# Autodesk Inventor assembly: BaseAssemblyMk1
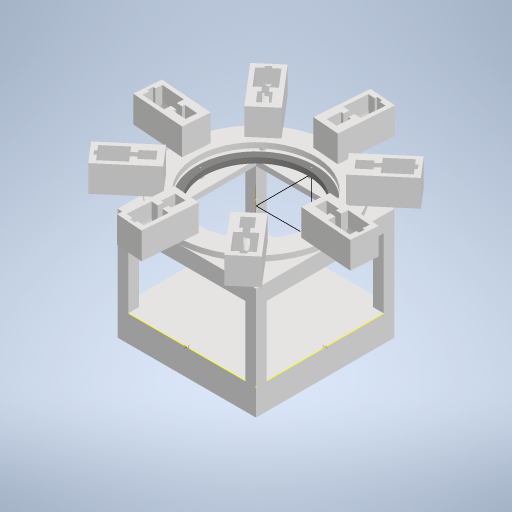
[picture p0: Inventor's stored thumbnail of the model, 512x512]
Saved by Autodesk Inventor 2023 (Build 270158000, 158)
## iProperties
Created: 2023-03-23
Part Number: BaseAssemblyMk1
Document SubType Name: Assembly
Designer: czapa
Author: czapa
## Documents named in this file (6)
- C:\Users\czapa\OneDrive\Documents\GitHub\S.P.I.C.E\3D Models\Version1\BaseAssemblyMk1.iam
- C:\Users\czapa\OneDrive\Documents\GitHub\S.P.I.C.E\3D Models\Version1\BaseMk1.ipt
- C:\Users\czapa\OneDrive\Documents\GitHub\S.P.I.C.E\3D Models\Version1\InnerBearingTable.ipt
- C:\Users\czapa\OneDrive\Documents\GitHub\S.P.I.C.E\3D Models\Version1\OuterBearingTable.ipt
- C:\Users\czapa\OneDrive\Documents\GitHub\S.P.I.C.E\3D Models\Version1\TableCover.ipt
- C:\Users\czapa\OneDrive\Documents\GitHub\S.P.I.C.E\3D Models\dcmotor_housing.ipt
## Components (12 placed, 5 different names)
1. BaseMk1:1 — Mate:1, Mate:2, Mate:3
2. InnerBearingTable:1 — Mate:1, Mate:2, Mate:3, Mate:4, Flush:1
3. OuterBearingTable:1 — Mate:4, Flush:1, Mate:5, Mate:6, Mate:7
4. TableCover:1 — Mate:5, Mate:6, Mate:7, Mate:8, Mate:9, Mate:10, Flush:2, Flush:3, Flush:4, Flush:5, Flush:6, Flush:7, Flush:8, Mate:11, Mate:12, Mate:13, Mate:14, Mate:15, Mate:16, Mate:17, Mate:18, Mate:19, Mate:20, Mate:21, Mate:22, Mate:23, Mate:24
5. dcmotor_housing:1 — Mate:8, Mate:9, Mate:10
6. dcmotor_housing:2 — Flush:2, Mate:11, Mate:18
7. dcmotor_housing:3 — Flush:5, Mate:12, Mate:21
8. dcmotor_housing:4 — Flush:8, Mate:14, Mate:19
9. dcmotor_housing:5 — Flush:6, Mate:16, Mate:22
10. dcmotor_housing:6 — Flush:3, Mate:13, Mate:23
11. dcmotor_housing:7 — Flush:4, Mate:17, Mate:20
12. dcmotor_housing:8 — Flush:7, Mate:15, Mate:24
## Relationships (32: Mate 24, Flush 8)
- Mate:1: BaseMk1:1 ↔ InnerBearingTable:1
- Mate:2: BaseMk1:1 ↔ InnerBearingTable:1
- Mate:3: BaseMk1:1 ↔ InnerBearingTable:1
- Mate:4: InnerBearingTable:1 ↔ OuterBearingTable:1
- Flush:1: InnerBearingTable:1 ↔ OuterBearingTable:1
- Mate:5: OuterBearingTable:1 ↔ TableCover:1
- Mate:6: OuterBearingTable:1 ↔ TableCover:1
- Mate:7: OuterBearingTable:1 ↔ TableCover:1
- Mate:8: TableCover:1 ↔ dcmotor_housing:1
- Mate:9: TableCover:1 ↔ dcmotor_housing:1
- Mate:10: TableCover:1 ↔ dcmotor_housing:1
- Flush:2: TableCover:1 ↔ dcmotor_housing:2
- Flush:3: TableCover:1 ↔ dcmotor_housing:6
- Flush:4: TableCover:1 ↔ dcmotor_housing:7
- Flush:5: TableCover:1 ↔ dcmotor_housing:3
- Flush:6: TableCover:1 ↔ dcmotor_housing:5
- Flush:7: TableCover:1 ↔ dcmotor_housing:8
- Flush:8: TableCover:1 ↔ dcmotor_housing:4
- Mate:11: TableCover:1 ↔ dcmotor_housing:2
- Mate:12: TableCover:1 ↔ dcmotor_housing:3
- Mate:13: TableCover:1 ↔ dcmotor_housing:6
- Mate:14: TableCover:1 ↔ dcmotor_housing:4
- Mate:15: TableCover:1 ↔ dcmotor_housing:8
- Mate:16: TableCover:1 ↔ dcmotor_housing:5
- Mate:17: TableCover:1 ↔ dcmotor_housing:7
- Mate:18: TableCover:1 ↔ dcmotor_housing:2
- Mate:19: TableCover:1 ↔ dcmotor_housing:4
- Mate:20: TableCover:1 ↔ dcmotor_housing:7
- Mate:21: TableCover:1 ↔ dcmotor_housing:3
- Mate:22: TableCover:1 ↔ dcmotor_housing:5
- Mate:23: TableCover:1 ↔ dcmotor_housing:6
- Mate:24: TableCover:1 ↔ dcmotor_housing:8
